# Autodesk Inventor assembly: LargeFinderEyepieces
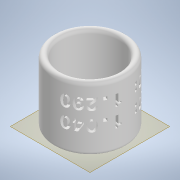
[picture p0: Inventor's stored thumbnail of the model, 180x180]
Saved by Autodesk Inventor 2021.1 (Build 251245000, 245)
## iProperties
Created: 2020-09-27
Part Number: LargeFinderEyepieces
Document SubType Name: Assembly
Designer: robst
Author: robst
## Documents named in this file (2)
- C:\git\CAD-Development\robSteele\TelescopeProjects\LensCovers\LargeFinderEyepieces.iam
- C:\git\CAD-Development\robSteele\TelescopeProjects\LensCovers\LargeFinderEyePieceCover.ipt
## Components (1 placed, 1 different names)
1. LargeFinderEyePieceCover:1 — Mate:1, Flush:1, Flush:2
## Relationships (3: Flush 2, Mate 1)
- Mate:1: LargeFinderEyePieceCover:1
- Flush:1: LargeFinderEyePieceCover:1
- Flush:2: LargeFinderEyePieceCover:1
